# Autodesk Inventor assembly: Graphics
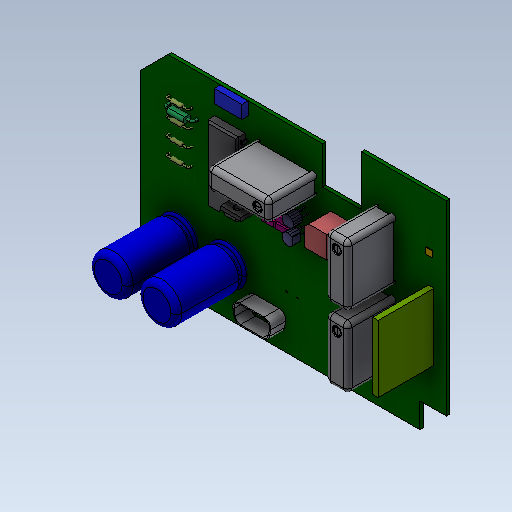
[picture p0: Inventor's stored thumbnail of the model, 512x512]
Saved by Autodesk Inventor 2020.1 (Build 241239000, 239)
## iProperties
Part Number: Graphics
Document SubType Name: Assembly
Created: 2003-04-02
Designer: t_enrig
Manufacturer: Standard
Standards Organization: Custom
Mass: 60.3399 g
Surface Area: 445.616 cm^2
Volume: 60.3399 cm^3
Density: 1 g/cm^3
Control State: 0
Master: False
Checked Out: False
Shininess: 64.0
Length Units: 11272
Angle Units: 11279
Time Units: 11290
Mass Units: 11286
Length Display Precision: 3
Angle Display Precision: 2
Compacted: True
Density: 0.0
Volumn: 0.0
Area: 0.0
PropertySet Name: Model Information
Author: t_enrig
## Documents named in this file (14)
- C:\Users\thom_tremblay\Desktop\Inventor ACP prep data\Week 1\Electrical Enclosure\Graphics.iam
- C:\Users\thom_tremblay\Desktop\Inventor ACP prep data\Week 1\Electrical Enclosure\RAD1100X390X870P89043.ipt
- C:\Users\thom_tremblay\Desktop\Inventor ACP prep data\Week 1\Electrical Enclosure\CPCYLD700X1400P30043.ipt
- C:\Users\thom_tremblay\Desktop\Inventor ACP prep data\Week 1\Electrical Enclosure\SMC_1206.ipt
- C:\Users\thom_tremblay\Desktop\Inventor ACP prep data\Week 1\Electrical Enclosure\DIP10024W600L1300.ipt
- C:\Users\thom_tremblay\Desktop\Inventor ACP prep data\Week 1\Electrical Enclosure\TO220.ipt
- C:\Users\thom_tremblay\Desktop\Inventor ACP prep data\Week 1\Electrical Enclosure\example1.ipt
- C:\Users\thom_tremblay\Desktop\Inventor ACP prep data\Week 1\Electrical Enclosure\CONP100VHTM1SQW10012K.ipt
- C:\Users\thom_tremblay\Desktop\Inventor ACP prep data\Week 1\Electrical Enclosure\DAXD100P40043.ipt
- C:\Users\thom_tremblay\Desktop\Inventor ACP prep data\Week 1\Electrical Enclosure\LTP.ipt
- C:\Users\thom_tremblay\Desktop\Inventor ACP prep data\Week 1\Electrical Enclosure\DAXD150P50051.ipt
- C:\Users\thom_tremblay\Desktop\Inventor ACP prep data\Week 1\Electrical Enclosure\TO237.ipt
- C:\Users\thom_tremblay\Desktop\Inventor ACP prep data\Week 1\Electrical Enclosure\BR400X400X400P200X20043.ipt
- C:\Users\thom_tremblay\Desktop\Inventor ACP prep data\Week 1\Electrical Enclosure\FIDMARK2.ipt
## Components (23 placed, 13 different names)
1. RAD1100X390X870P89043
2. CPCYLD700X1400P30043
3. SMC_1206
4. DIP10024W600L1300
5. RAD1100X390X870P89043
6. TO220
7. example1
8. CONP100VHTM1SQW10012K
9. SMC_1206
10. DAXD150P50051
11. TO237
12. SMC_1206
13. CPCYLD700X1400P30043
14. RAD1100X390X870P89043
15. BR400X400X400P200X20043
16. FIDMARK2
17. TO237
18. SMC_1206
19. LTP:1
20. DAXD100P40043
21. DAXD100P40043:2
22. DAXD100P40043:3
23. DAXD100P40043:4
## Component patterns: (4 elements, first: DAXD100P40043)
